# Autodesk Inventor assembly: biggearsmallgearMIDDLESPACER
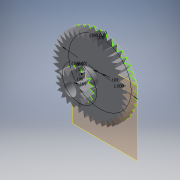
[picture p0: Inventor's stored thumbnail of the model, 180x180]
Saved by Autodesk Inventor 2018 (Build 220112000, 112)
## iProperties
Created: 2019-03-12
Part Number: biggearsmallgearMIDDLESPACER
Document SubType Name: Assembly
Designer: F8PLTW
Author: F8PLTW
## Documents named in this file (4)
- D:\biggearsmallgearMIDDLESPACER.iam
- D:\phonegearfinalBIG.ipt
- D:\phonecasespacer.ipt
- D:\phonecasegearSMALL.ipt
## Components (3 placed, 3 different names)
1. phonegearfinalBIG:1 — Mate:1, Mate:2
2. phonecasespacer:1 — Mate:1, Mate:2, Mate:3, Mate:4
3. phonecasegearSMALL:1 — Mate:3, Mate:4
## Relationships (4: Mate 4)
- Mate:1: phonegearfinalBIG:1 ↔ phonecasespacer:1
- Mate:2: phonegearfinalBIG:1 ↔ phonecasespacer:1
- Mate:3: phonecasespacer:1 ↔ phonecasegearSMALL:1
- Mate:4: phonecasespacer:1 ↔ phonecasegearSMALL:1
